# Autodesk Inventor assembly: Motor assembly
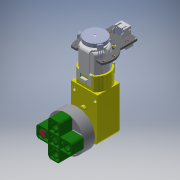
[picture p0: Inventor's stored thumbnail of the model, 180x180]
Saved by Autodesk Inventor 2019 (Build 230136000, 136)
## iProperties
Created: 2018-11-22
Part Number: Motor assembly
Document SubType Name: Assembly
Designer: Varga Daniel
Author: Varga Daniel
## Documents named in this file (5)
- C:\!_Dani\!_cloud\OneDrive\!_munka\Revolution\RevvyDemoKit\Structural parts\Demo parts\Motor\Motor assembly.iam
- C:\!_Dani\!_cloud\OneDrive\!_munka\Revolution\RevvyDemoKit\Structural parts\Demo parts\Motor\FIT0450 motor\FIT0450.iam
- C:\!_Dani\!_cloud\OneDrive\!_munka\Revolution\RevvyDemoKit\Structural parts\Connetor Pins\cp1x1.ipt
- C:\!_Dani\!_cloud\OneDrive\!_munka\Revolution\RevvyDemoKit\Structural parts\Axle Connectors\Axle connector 3x3 cross.ipt
- C:\!_Dani\!_cloud\OneDrive\!_munka\Revolution\RevvyDemoKit\Structural parts\Demo parts\Motor\Motor rotor.ipt
## Components (4 placed, 4 different names)
1. FIT0450:1 [sub-assembly] — Mate:7, Angle:1, Mate:8
2. cp1x1:1 — Mate:2, Mate:3, Mate:4, Mate:5
3. Axle connector 3x3 cross:1 — Mate:2, Mate:3, Mate:6
4. Motor rotor:1 — Mate:4, Mate:5, Mate:6, Mate:7, Angle:1, Mate:8
## Relationships (8: Mate 7, Angle 1)
- Mate:2: cp1x1:1 ↔ Axle connector 3x3 cross:1
- Mate:3: cp1x1:1 ↔ Axle connector 3x3 cross:1
- Mate:4: cp1x1:1 ↔ Motor rotor:1
- Mate:5: cp1x1:1 ↔ Motor rotor:1
- Mate:6: Axle connector 3x3 cross:1 ↔ Motor rotor:1
- Mate:7: FIT0450:1 ↔ Motor rotor:1
- Angle:1 (0 deg): FIT0450:1 ↔ Motor rotor:1
- Mate:8: FIT0450:1 ↔ Motor rotor:1
